# Autodesk Inventor assembly: VerticalSlides2.2
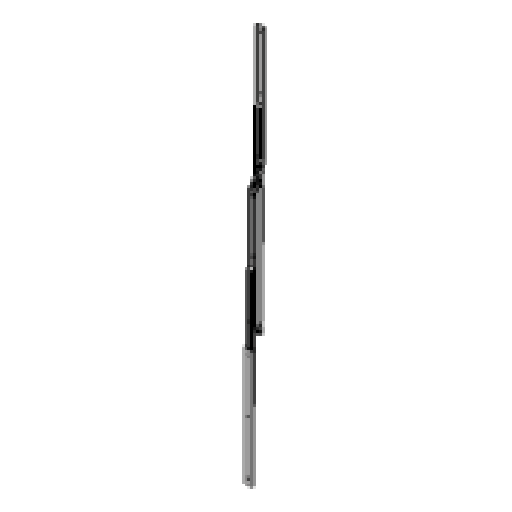
[picture p0: Inventor's stored thumbnail of the model, 512x512]
Saved by Autodesk Inventor 2023 (Build 270158000, 158)
## iProperties
Created: 2022-09-10
Part Number: VerticalSlides2.2
Document SubType Name: Assembly
Designer: deli
Author: deli
## Documents named in this file (5)
- C:\Users\deli\OneDrive - Eastside Preparatory School\FTC\8103-power-play\CAD\VerticalSlides2.2.iam
- C:\Users\deli\OneDrive - Eastside Preparatory School\FTC\8103-power-play\CAD\FTC-parts\KC-362-30.iam
- C:\Users\deli\OneDrive - Eastside Preparatory School\FTC\8103-power-play\CAD\VerticalSlideMiddleBottom2.2.ipt
- C:\Users\deli\OneDrive - Eastside Preparatory School\FTC\8103-power-play\CAD\VerticalSlideMiddleTop2.2.ipt
- C:\Users\deli\OneDrive - Eastside Preparatory School\FTC\8103-power-play\CAD\FTC-parts\LongRobotics\3x12x4mm-bearing.ipt
## Components (6 placed, 4 different names)
1. KC-362-30:2 [sub-assembly] — Mate:1, Mate:5, Mate:6, Mate:10, Mate:13
2. KC-362-30:3 [sub-assembly] — Mate:12, Mate:14, Mate:15, Mate:16
3. VerticalSlideMiddleBottom2.2:1 — Mate:6, Mate:10, Mate:12, Mate:16, Mate:17, Mate:18
4. VerticalSlideMiddleTop2.2:1 — Mate:1, Mate:5, Mate:13, Mate:14, Mate:15, Mate:19, Mate:20
5. 3x12x4mm-bearing:1 — Mate:19, Mate:20
6. 3x12x4mm-bearing:2 — Mate:17, Mate:18
## Relationships (13: Mate 13)
- Mate:1: KC-362-30:2 ↔ VerticalSlideMiddleTop2.2:1
- Mate:5: KC-362-30:2 ↔ VerticalSlideMiddleTop2.2:1
- Mate:6: KC-362-30:2 ↔ VerticalSlideMiddleBottom2.2:1
- Mate:10: KC-362-30:2 ↔ VerticalSlideMiddleBottom2.2:1
- Mate:12: KC-362-30:3 ↔ VerticalSlideMiddleBottom2.2:1
- Mate:13: KC-362-30:2 ↔ VerticalSlideMiddleTop2.2:1
- Mate:14: KC-362-30:3 ↔ VerticalSlideMiddleTop2.2:1
- Mate:15: KC-362-30:3 ↔ VerticalSlideMiddleTop2.2:1
- Mate:16: KC-362-30:3 ↔ VerticalSlideMiddleBottom2.2:1
- Mate:17 (0.25 mm): VerticalSlideMiddleBottom2.2:1 ↔ 3x12x4mm-bearing:2
- Mate:18: VerticalSlideMiddleBottom2.2:1 ↔ 3x12x4mm-bearing:2
- Mate:19 (0.25 mm): VerticalSlideMiddleTop2.2:1 ↔ 3x12x4mm-bearing:1
- Mate:20: VerticalSlideMiddleTop2.2:1 ↔ 3x12x4mm-bearing:1
